# Autodesk Inventor assembly: Screwdriver Assy
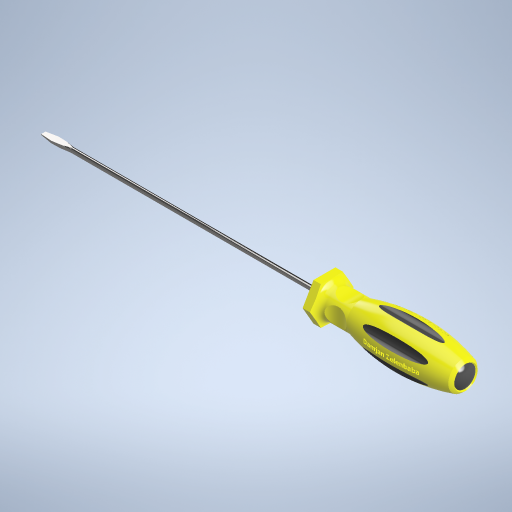
[picture p0: Inventor's stored thumbnail of the model, 512x512]
Saved by Autodesk Inventor 2024 (Build 280153000, 153)
## iProperties
Created: 2023-06-13
Part Number: Screwdriver Assy
Document SubType Name: Assembly
Designer: 69
Author: 69
## Documents named in this file (3)
- C:\Users\69\Desktop\git new\Flat Head Screwdriver\Screwdriver Assy.iam
- C:\Users\69\Desktop\git new\Flat Head Screwdriver\Handle.ipt
- C:\Users\69\Desktop\git new\Flat Head Screwdriver\Shaft.ipt
## Components (2 placed, 2 different names)
1. Handle:1 — Mate:1, Insert:1
2. Shaft:1 — Mate:1, Insert:1
## Relationships (2: Mate 1, Insert 1)
- Mate:1: Handle:1 ↔ Shaft:1
- Insert:1: Handle:1 ↔ Shaft:1
